# Autodesk Inventor assembly: Synchronous Belts Transmission
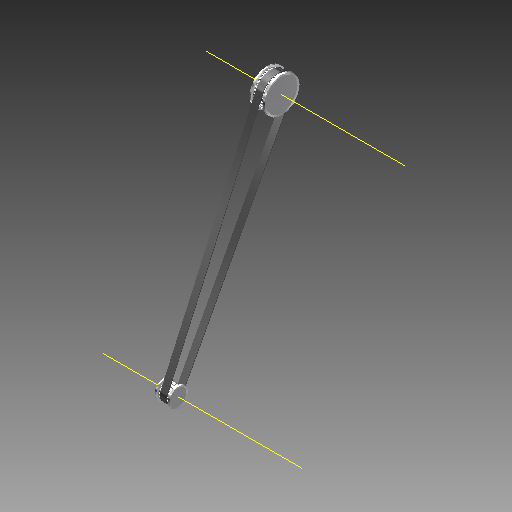
[picture p0: Inventor's stored thumbnail of the model, 512x512]
Saved by Autodesk Inventor 2019.4 (Build 234330000, 330)
## iProperties
Created: 2020-02-16
Part Number: Synchronous Belts Transmission
Document SubType Name: Assembly
Designer: admin
Mass: 289.286 g
Surface Area: 290.48 cm^2
Volume: 43.904 cm^3
Density: 6.58907 g/cm^3
ClientObjectVersion: 1
Author: admin
## Documents named in this file (4)
- C:\Users\Mark\Desktop\7738 Helion Engineering\7738-2020\Robot V2\Turret\Turret Assembly\Design Accelerator\Synchronous Belts Transmission11.iam
- C:\Users\Mark\Desktop\7738 Helion Engineering\7738-2020\Robot V2\Turret\Turret Assembly\Design Accelerator\Synchronous Belt11.ipt
- C:\Users\Mark\Desktop\7738 Helion Engineering\7738-2020\Robot V2\Turret\Turret Assembly\Design Accelerator\Synchronous Pulley111.ipt
- C:\Users\Mark\Desktop\7738 Helion Engineering\7738-2020\Robot V2\Turret\Turret Assembly\Design Accelerator\Synchronous Pulley211.ipt
## Components (3 placed, 3 different names)
1. Synchronous Belt:1 — Flush:1, Mate:1, Mate:2, Flush:2, Mate:3, Mate:4
2. Synchronous Pulley1:1 — Flush:1, Mate:1, Mate:2, Rotation:1
3. Synchronous Pulley2:1 — Flush:2, Mate:3, Rotation:1, Mate:4
## Relationships (7: Mate 4, Flush 2, RelateRotation 1)
- Flush:1: Synchronous Belt:1 ↔ Synchronous Pulley1:1
- Mate:1: Synchronous Belt:1 ↔ Synchronous Pulley1:1
- Mate:2: Synchronous Belt:1 ↔ Synchronous Pulley1:1
- Flush:2: Synchronous Belt:1 ↔ Synchronous Pulley2:1
- Mate:3: Synchronous Belt:1 ↔ Synchronous Pulley2:1
- Rotation:1 [RelateRotation] (0.5 ul): Synchronous Pulley1:1 ↔ Synchronous Pulley2:1
- Mate:4: Synchronous Belt:1 ↔ Synchronous Pulley2:1
